# Autodesk Inventor assembly: A2017_T5_06
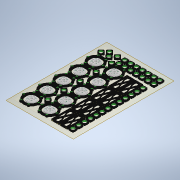
[picture p0: Inventor's stored thumbnail of the model, 180x180]
Saved by Autodesk Inventor 2022 (Build 260153000, 153)
## iProperties
Created: 2022-09-28
Part Number: A2017_T5_06
Document SubType Name: Assembly
Designer: Masato
Author: Masato
## Documents named in this file (6)
- C:\Users\ヨコオリク\Documents\CITBrains\SUSTAINA-OP\Cam\A2017_T5\A2017_T5_06.iam
- C:\Users\ヨコオリク\Documents\CITBrains\SUSTAINA-OP\Cam\DisposableBoard.ipt
- C:\Users\ヨコオリク\Documents\CITBrains\SUSTAINA-OP\LowerBody\Knee\Knee_clamp.ipt
- C:\Users\ヨコオリク\Documents\CITBrains\SUSTAINA-OP\LowerBody\Link\BackLink_diagonal.ipt
- C:\Users\ヨコオリク\Documents\CITBrains\SUSTAINA-OP\UpperBody\Trunk\CrossRollerBearing\Inner_support_stand.ipt
- C:\Users\ヨコオリク\Documents\CITBrains\SUSTAINA-OP\UpperBody\Trunk\CrossRollerBearing\Outer_support_stand.ipt
## Components (65 placed, 5 different names)
1. DisposableBoard:1 — フラッシュ:1, フラッシュ:2, フラッシュ:3, フラッシュ:4, 正接:1, 正接:2, フラッシュ:7, 正接:6, 正接:7, 正接:9, メイト:12, 正接:10, 正接:11
2. Knee_clamp:5 — メイト:7
3. Inner_support_stand:1 — メイト:2, 挿入:1, 角度:2
4. Outer_support_stand:1 — メイト:1, 角度:1, 正接:1, 正接:2, 挿入:1
5. Inner_support_stand:2
6. Outer_support_stand:2 — 正接:4
7. Inner_support_stand:3
8. Outer_support_stand:3
9. Inner_support_stand:4
10. Outer_support_stand:4
11. Inner_support_stand:5
12. Outer_support_stand:5
13. Inner_support_stand:6
14. Outer_support_stand:6
15. Inner_support_stand:7
16. Outer_support_stand:7
17. Inner_support_stand:8
18. Outer_support_stand:8
19. Inner_support_stand:9
20. Outer_support_stand:9 — 正接:8
21. Inner_support_stand:10
22. Outer_support_stand:10
23. Knee_clamp:1 — メイト:4, メイト:5, メイト:6
24. Knee_clamp:2
25. Knee_clamp:3
26. Knee_clamp:4
27. BackLink_diagonal:2 — メイト:8, フラッシュ:7, 正接:4
28. BackLink_diagonal:3 — 正接:5
29. BackLink_diagonal:4
30. BackLink_diagonal:5
31. BackLink_diagonal:6
32. BackLink_diagonal:7
33. BackLink_diagonal:8
34. BackLink_diagonal:9
35. Knee_clamp:6 — メイト:9, 角度:3, 正接:5, 正接:6
36. Knee_clamp:7
37. Knee_clamp:8
38. Knee_clamp:9
39. Knee_clamp:10
40. Knee_clamp:11
41. Knee_clamp:12
42. Knee_clamp:13
43. Knee_clamp:14
44. Knee_clamp:15
45. Knee_clamp:16
46. Knee_clamp:17
47. Knee_clamp:18
48. Knee_clamp:21 — メイト:10, 角度:4, 正接:7, 正接:8
49. Knee_clamp:22 — メイト:11, 角度:5, 正接:9, メイト:12
50. Knee_clamp:23
51. Knee_clamp:24
52. Knee_clamp:25 — メイト:13, 角度:6, 正接:10, 正接:11
53. Knee_clamp:26
54. Knee_clamp:27
55. Knee_clamp:28
56. Knee_clamp:29
57. Knee_clamp:30
58. Knee_clamp:31
59. Knee_clamp:32
60. Knee_clamp:33
61. Knee_clamp:34
62. Knee_clamp:35
63. Knee_clamp:36
64. Knee_clamp:37
65. Knee_clamp:38
## Component patterns: (10 elements, first: Inner_support_stand:1 + Outer_support_stand:1), (4 elements, first: Knee_clamp:1), (8 elements, first: BackLink_diagonal:2), (13 elements, first: Knee_clamp:6), (2 elements, first: Knee_clamp:21 + Knee_clamp:22), (14 elements, first: Knee_clamp:25)
## Relationships (34: Mate 12, Tangent 10, Angle 6, Flush 5, Insert 1)
- フラッシュ:1 [Flush]: DisposableBoard:1
- フラッシュ:2 [Flush]: DisposableBoard:1
- フラッシュ:3 [Flush]: DisposableBoard:1
- フラッシュ:4 [Flush]: DisposableBoard:1
- メイト:1 [Mate]: Outer_support_stand:1
- メイト:2 [Mate]: Inner_support_stand:1
- メイト:4 [Mate]: Knee_clamp:1
- 角度:1 [Angle] (90 deg): Outer_support_stand:1
- 正接:1 [Tangent] (2 mm): DisposableBoard:1 ↔ Outer_support_stand:1
- 正接:2 [Tangent] (2 mm): DisposableBoard:1 ↔ Outer_support_stand:1
- 挿入:1 [Insert]: Inner_support_stand:1 ↔ Outer_support_stand:1
- 角度:2 [Angle] (0 deg): Inner_support_stand:1
- メイト:5 [Mate] (60.5 mm): Knee_clamp:1
- メイト:6 [Mate] (51.568 mm): Knee_clamp:1
- メイト:7 [Mate] (60.5 mm): Knee_clamp:5
- メイト:8 [Mate]: BackLink_diagonal:2
- フラッシュ:7 [Flush] (2 mm): DisposableBoard:1 ↔ BackLink_diagonal:2
- 正接:4 [Tangent] (2.1 mm): Outer_support_stand:2 ↔ BackLink_diagonal:2
- メイト:9 [Mate]: Knee_clamp:6
- 角度:3 [Angle] (45 deg): Knee_clamp:6
- 正接:5 [Tangent] (2.1 mm): BackLink_diagonal:3 ↔ Knee_clamp:6
- 正接:6 [Tangent] (2 mm): DisposableBoard:1 ↔ Knee_clamp:6
- メイト:10 [Mate]: Knee_clamp:21
- 角度:4 [Angle] (0 deg): Knee_clamp:21
- 正接:7 [Tangent] (2 mm): DisposableBoard:1 ↔ Knee_clamp:21
- 正接:8 [Tangent] (2.1 mm): Outer_support_stand:9 ↔ Knee_clamp:21
- メイト:11 [Mate]: Knee_clamp:22
- 角度:5 [Angle] (0 deg): Knee_clamp:22
- 正接:9 [Tangent] (2.1 mm): DisposableBoard:1 ↔ Knee_clamp:22
- メイト:12 [Mate] (-26.5 mm): DisposableBoard:1 ↔ Knee_clamp:22
- メイト:13 [Mate]: Knee_clamp:25
- 角度:6 [Angle] (45 deg): Knee_clamp:25
- 正接:10 [Tangent] (2 mm): DisposableBoard:1 ↔ Knee_clamp:25
- 正接:11 [Tangent] (2.5 mm): DisposableBoard:1 ↔ Knee_clamp:25
